# Autodesk Inventor assembly: gasienica_zlozenie_final
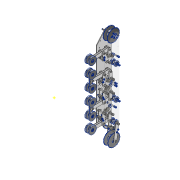
[picture p0: Inventor's stored thumbnail of the model, 180x180]
Saved by Autodesk Inventor 2020.3 (Build 243373000, 373)
## iProperties
Created: 2021-10-24
Part Number: gasienica_zlozenie_final
Document SubType Name: Assembly
Designer: Patryk Szydlik
Project: Projekt gąsienicowego układu jezdnego robota mobilnego "Ariadna"
Description: Projekt gąsienicowego układu jezdnego robota mobilnego "Ariadna"
Author: Patryk Szydlik
Title: Projekt gąsienicowego układu jezdnego robota mobilnego "Ariadna"
Subject: Projekt gąsienicowego układu jezdnego robota mobilnego "Ariadna"
## Documents named in this file (15)
- C:\Users\patry\Desktop\Semestr 7\Inzynierka\Projekt inventor\Ariadna_inzynierka\Workspaces\Obszar roboczy\Obszar roboczy\Naped\Zawieszenie_v3\gasienica_zlozenie_final.iam
- C:\Users\patry\Desktop\Semestr 7\Inzynierka\Projekt inventor\Ariadna_inzynierka\Workspaces\Obszar roboczy\Obszar roboczy\Naped\Sruby\M8_nut_6.5mm_MIR1.ipt
- C:\Users\patry\Desktop\Semestr 7\Inzynierka\Projekt inventor\Ariadna_inzynierka\Workspaces\Obszar roboczy\Obszar roboczy\Naped\Sruby\M8x80_threaded_MIR1.ipt
- C:\Users\patry\Desktop\Semestr 7\Inzynierka\Projekt inventor\Ariadna_inzynierka\Workspaces\Obszar roboczy\Obszar roboczy\Naped\Sruby\M8_pad_MIR1.ipt
- C:\Users\patry\Desktop\Semestr 7\Inzynierka\Projekt inventor\Ariadna_inzynierka\Workspaces\Obszar roboczy\Obszar roboczy\Naped\Lozyska\608ZZ-8mm\bearings-608zz-80018-1.snapshot.1\608zz_MIR1.ipt
- C:\Users\patry\Desktop\Semestr 7\Inzynierka\Projekt inventor\Ariadna_inzynierka\Workspaces\Obszar roboczy\Obszar roboczy\Naped\Kola\kolo_napedowe.iam
- C:\Users\patry\Desktop\Semestr 7\Inzynierka\Projekt inventor\Ariadna_inzynierka\Workspaces\Obszar roboczy\Obszar roboczy\Naped\Kola\holder_wheel_pair.iam
- C:\Users\patry\Desktop\Semestr 7\Inzynierka\Projekt inventor\Ariadna_inzynierka\Workspaces\Obszar roboczy\Obszar roboczy\Naped\Zawieszenie_v3\plyta_boczna.ipt
- C:\Users\patry\Desktop\Semestr 7\Inzynierka\Projekt inventor\Ariadna_inzynierka\Workspaces\Obszar roboczy\Obszar roboczy\Naped\Kola\single_wheel_dummie.iam
- C:\Users\patry\Desktop\Semestr 7\Inzynierka\Projekt inventor\Ariadna_inzynierka\Workspaces\Obszar roboczy\Obszar roboczy\Naped\Sruby\tuleja_M5_M10_15.ipt
- C:\Users\patry\Desktop\Semestr 7\Inzynierka\Projekt inventor\Ariadna_inzynierka\Workspaces\Obszar roboczy\Obszar roboczy\Naped\Sruby\tuleja_M6_M10_7,5.ipt
- C:\Users\patry\Desktop\Semestr 7\Inzynierka\Projekt inventor\Ariadna_inzynierka\Workspaces\Obszar roboczy\Obszar roboczy\Naped\Zawieszenie_v3\napinacz_zlozenie_final.iam
- C:\Users\patry\Desktop\Semestr 7\Inzynierka\Projekt inventor\Ariadna_inzynierka\Workspaces\Obszar roboczy\Obszar roboczy\Naped\Zawieszenie_v3\wahacz_tylny_szkic.iam
- C:\Users\patry\Desktop\Semestr 7\Inzynierka\Projekt inventor\Ariadna_inzynierka\Workspaces\Obszar roboczy\Obszar roboczy\Naped\Zawieszenie_v3\wahacz_zewn_szkic.iam
- C:\Users\patry\Desktop\Semestr 7\Inzynierka\Projekt inventor\Ariadna_inzynierka\Workspaces\Obszar roboczy\Obszar roboczy\Naped\Zawieszenie_v3\wahacz_wewn_szkic.iam
## Components (25 placed, 14 different names)
1. M8_nut_6.5mm_MIR1:1
2. M8x80_threaded_MIR1:1
3. M8_nut_6.5mm_MIR1:2
4. M8_nut_6.5mm_MIR1:3
5. M8_pad_MIR1:1
6. M8_pad_MIR1:2
7. M8_pad_MIR1:3
8. M8_pad_MIR1:4
9. 608zz_MIR1:1
10. 608zz_MIR1:2 — Zestawiające:1077, Równoległe:74
11. kolo_napedowe:1 [sub-assembly]
12. holder_wheel_pair:4 [sub-assembly] — Zestawiające:1082, Zestawiające:1083
13. holder_wheel_pair:5 [sub-assembly] — Zestawiające:1081, Zestawiające:1084
14. plyta_boczna:1 — Zestawiające:1075, Zestawiające:1076, Zestawiające:1077, Zestawiające:1078, Równoległe:74, Kątowe:22, Zestawiające:1081, Zestawiające:1082, Zestawiające:1083, Zestawiające:1084, Zestawiające:1813, Zestawiające:1814, Zestawiające:1825, Zestawiające:1826, Zestawiające:1827, Zestawiające:1828, Zestawiające:1829, Zestawiające:1830, Zestawiające:1831, Zestawiające:1832, Zestawiające:1833, Zestawiające:1834, Zestawiające:1835, Zestawiające:1836
15. plyta_boczna:2 — Zestawiające:1075, Zestawiające:1076, Zestawiające:1078, Zestawiające:1812
16. napinacz_zlozenie_final:1 [sub-assembly] — Zestawiające:1812, Zestawiające:1813, Zestawiające:1814, Zestawiające:1823, Zestawiające:1824
17. single_wheel_dummie:1 [sub-assembly] — Zestawiające:1820, Zestawiające:1821, Zestawiające:1822
18. single_wheel_dummie:2 [sub-assembly]
19. tuleja_M5_M10_15:1
20. tuleja_M6_M10_7,5:1 — Zestawiające:1821, Zestawiające:1823
21. tuleja_M6_M10_7,5:2 — Zestawiające:1820, Zestawiające:1822, Zestawiające:1824
22. wahacz_tylny_szkic:1 [sub-assembly] — Zestawiające:1825, Zestawiające:1826, Zestawiające:1827
23. wahacz_zewn_szkic:1 [sub-assembly] — Zestawiające:1828, Zestawiające:1829, Zestawiające:1830
24. wahacz_wewn_szkic:1 [sub-assembly] — Zestawiające:1831, Zestawiające:1832, Zestawiające:1833
25. wahacz_wewn_szkic:2 [sub-assembly] — Zestawiające:1834, Zestawiające:1835, Zestawiające:1836
## Relationships (55: Mate 53, Flush 1, Angle 1)
- [Mate]: M8_nut_6.5mm_MIR1:1 ↔ M8x80_threaded_MIR1:1
- [Mate]: M8x80_threaded_MIR1:1 ↔ M8_nut_6.5mm_MIR1:2
- [Mate]: M8x80_threaded_MIR1:1 ↔ M8_nut_6.5mm_MIR1:3
- [Mate]: M8_nut_6.5mm_MIR1:1 ↔ M8_pad_MIR1:1
- [Mate] (7 mm): M8x80_threaded_MIR1:1 ↔ M8_pad_MIR1:1
- [Mate]: M8x80_threaded_MIR1:1 ↔ M8_pad_MIR1:1
- [Mate]: M8_nut_6.5mm_MIR1:1 ↔ M8_pad_MIR1:2
- [Mate]: M8x80_threaded_MIR1:1 ↔ M8_pad_MIR1:2
- [Mate] (7 mm): M8_nut_6.5mm_MIR1:2 ↔ M8_pad_MIR1:3
- [Mate]: M8_nut_6.5mm_MIR1:3 ↔ M8_pad_MIR1:3
- [Mate]: M8x80_threaded_MIR1:1 ↔ M8_pad_MIR1:3
- [Mate]: M8_nut_6.5mm_MIR1:3 ↔ M8_pad_MIR1:4
- [Mate] (31 mm): M8_pad_MIR1:2 ↔ M8_pad_MIR1:4
- [Mate]: M8x80_threaded_MIR1:1 ↔ M8_pad_MIR1:4
- [Mate]: M8x80_threaded_MIR1:1 ↔ 608zz_MIR1:1
- [Mate]: M8_nut_6.5mm_MIR1:2 ↔ 608zz_MIR1:1
- [Mate]: M8x80_threaded_MIR1:1 ↔ 608zz_MIR1:2
- [Mate]: M8x80_threaded_MIR1:1 ↔ 608zz_MIR1:2
- [Mate]: M8x80_threaded_MIR1:1 ↔ kolo_napedowe:1
- [Mate]: M8_pad_MIR1:2 ↔ kolo_napedowe:1
- Zestawiające:1075 [Mate]: plyta_boczna:1 ↔ plyta_boczna:2
- Zestawiające:1076 [Mate]: plyta_boczna:1 ↔ plyta_boczna:2
- Zestawiające:1077 [Mate]: 608zz_MIR1:2 ↔ plyta_boczna:1
- Zestawiające:1078 [Mate] (50 mm): plyta_boczna:1 ↔ plyta_boczna:2
- Równoległe:74 [Flush] (-1 mm): 608zz_MIR1:2 ↔ plyta_boczna:1
- Kątowe:22 [Angle] (180 deg): plyta_boczna:1
- Zestawiające:1081 [Mate]: holder_wheel_pair:5 ↔ plyta_boczna:1
- Zestawiające:1082 [Mate]: holder_wheel_pair:4 ↔ plyta_boczna:1
- Zestawiające:1083 [Mate]: holder_wheel_pair:4 ↔ plyta_boczna:1
- Zestawiające:1084 [Mate]: holder_wheel_pair:5 ↔ plyta_boczna:1
- Zestawiające:1812 [Mate]: plyta_boczna:2 ↔ napinacz_zlozenie_final:1
- Zestawiające:1813 [Mate]: plyta_boczna:1 ↔ napinacz_zlozenie_final:1
- Zestawiające:1814 [Mate] (0.043 mm): plyta_boczna:1 ↔ napinacz_zlozenie_final:1
- [Mate]: single_wheel_dummie:1 ↔ tuleja_M5_M10_15:1
- [Mate]: single_wheel_dummie:1 ↔ tuleja_M5_M10_15:1
- [Mate]: single_wheel_dummie:2 ↔ tuleja_M5_M10_15:1
- [Mate]: single_wheel_dummie:2 ↔ tuleja_M5_M10_15:1
- [Mate]: single_wheel_dummie:2 ↔ tuleja_M6_M10_7,5:1
- Zestawiające:1820 [Mate]: single_wheel_dummie:1 ↔ tuleja_M6_M10_7,5:2
- Zestawiające:1821 [Mate]: single_wheel_dummie:1 ↔ tuleja_M6_M10_7,5:1
- Zestawiające:1822 [Mate]: single_wheel_dummie:1 ↔ tuleja_M6_M10_7,5:2
- Zestawiające:1823 [Mate]: napinacz_zlozenie_final:1 ↔ tuleja_M6_M10_7,5:1
- Zestawiające:1824 [Mate]: napinacz_zlozenie_final:1 ↔ tuleja_M6_M10_7,5:2
- Zestawiające:1825 [Mate]: plyta_boczna:1 ↔ wahacz_tylny_szkic:1
- Zestawiające:1826 [Mate]: plyta_boczna:1 ↔ wahacz_tylny_szkic:1
- Zestawiające:1827 [Mate]: plyta_boczna:1 ↔ wahacz_tylny_szkic:1
- Zestawiające:1828 [Mate]: plyta_boczna:1 ↔ wahacz_zewn_szkic:1
- Zestawiające:1829 [Mate]: plyta_boczna:1 ↔ wahacz_zewn_szkic:1
- Zestawiające:1830 [Mate] (0.05 mm): plyta_boczna:1 ↔ wahacz_zewn_szkic:1
- Zestawiające:1831 [Mate]: plyta_boczna:1 ↔ wahacz_wewn_szkic:1
- Zestawiające:1832 [Mate]: plyta_boczna:1 ↔ wahacz_wewn_szkic:1
- Zestawiające:1833 [Mate] (0.05 mm): plyta_boczna:1 ↔ wahacz_wewn_szkic:1
- Zestawiające:1834 [Mate]: plyta_boczna:1 ↔ wahacz_wewn_szkic:2
- Zestawiające:1835 [Mate]: plyta_boczna:1 ↔ wahacz_wewn_szkic:2
- Zestawiające:1836 [Mate] (0.05 mm): plyta_boczna:1 ↔ wahacz_wewn_szkic:2
## Named parameters: d102_d31 = 0 mm, d103_d32 = 7 mm, d104_d33 = 0 mm, d105_d34 = 0 mm, d705_d35 = 0 mm, d706_d36 = 31 mm, d707_d37 = 0 mm, d109_d23 = 0 mm, d110_d24 = 0 mm, d111_d25 = 0 mm, d112_d26 = 0 mm, d113_d27 = 7 mm, d114_d28 = 0 mm, d115_d30 = 0 mm, d715_d116 = 0 mm, d716_d117 = 0 mm, d717_d118 = 0 mm, d718_d119 = 0 mm, susp_angle = 90 deg, tlok_scisniety = -13 mm, tlok_wyprostowany = 1 mm, d2405_susp_angle = 90 deg, dR = 2 mm
